# Autodesk Inventor assembly: Tower
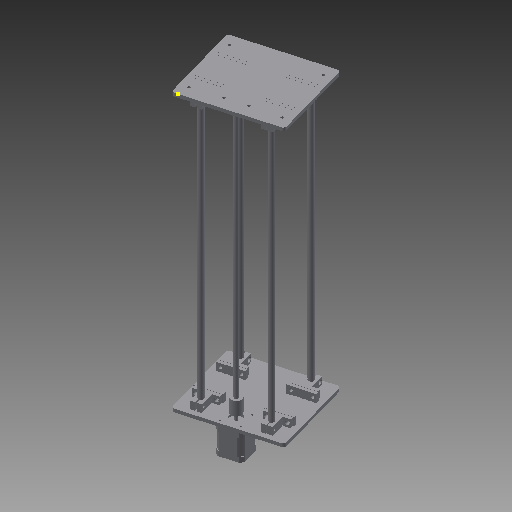
[picture p0: Inventor's stored thumbnail of the model, 512x512]
Saved by Autodesk Inventor 2019 (Build 230136000, 136)
## iProperties
Created: 2021-11-03
Part Number: Tower
Document SubType Name: Assembly
Designer: Mohamed
Author: Mohamed
## Documents named in this file (10)
- D:\mody\IndustrialLine\SortingAndStorage\Inventor\SSCARA Robot\Tower.iam
- D:\mody\IndustrialLine\SortingAndStorage\Inventor\SSCARA Robot\e_lead.ipt
- D:\mody\IndustrialLine\SortingAndStorage\Inventor\SSCARA Robot\e_coupler.ipt
- D:\mody\IndustrialLine\SortingAndStorage\Inventor\SSCARA Robot\e_circuler rod 400mm.ipt
- D:\mody\IndustrialLine\SortingAndStorage\Inventor\SSCARA Robot\e_top 1.ipt
- D:\mody\IndustrialLine\SortingAndStorage\Inventor\SSCARA Robot\e_linear rail support.ipt
- D:\mody\IndustrialLine\SortingAndStorage\Inventor\SSCARA Robot\nema 17 motor.ipt
- D:\mody\IndustrialLine\SortingAndStorage\Inventor\SSCARA Robot\e_rail support.ipt
- D:\mody\IndustrialLine\SortingAndStorage\Inventor\SSCARA Robot\e_k8_flanged bearing.iam
- D:\mody\IndustrialLine\SortingAndStorage\Inventor\SSCARA Robot\e_bot 1.ipt
## Components (26 placed, 9 different names)
1. e_top 1:1 — Mate:5, Mate:6, Mate:7, Mate:8, Mate:13, Flush:3, Flush:4, Flush:5, Flush:6, Mate:22, Mate:23, Mate:24, Mate:25, Mate:26, Mate:27, Mate:29, Mate:33, Mate:34, Mate:35, Mate:76, Mate:77
2. e_linear rail support:1 — Mate:5, Flush:1, Mate:14, Mate:19, Mate:30
3. e_linear rail support:2 — Mate:8, Flush:1, Mate:15, Mate:18, Mate:31
4. e_linear rail support:3 — Mate:7, Flush:2, Mate:17, Mate:21, Mate:32
5. e_linear rail support:4 — Mate:6, Flush:2, Mate:16, Mate:20, Mate:28
6. nema 17 motor:1 — Mate:13, Mate:38, Mate:39, Mate:76, Mate:77
7. e_rail support:1 — Flush:3, Mate:14, Mate:19, Mate:26, Mate:27
8. e_rail support:2 — Flush:4, Mate:15, Mate:18, Mate:25
9. e_rail support:3 — Flush:5, Mate:16, Mate:20, Mate:22, Mate:23
10. e_rail support:4 — Flush:6, Mate:17, Mate:21, Mate:24
11. e_circuler rod 400mm:1 — Mate:30, Mate:34, Mate:75
12. e_circuler rod 400mm:2 — Mate:31, Mate:33, Mate:79
13. e_circuler rod 400mm:3 — Mate:32, Mate:35, Mate:74
14. e_circuler rod 400mm:4 — Mate:28, Mate:29, Mate:73
15. e_coupler:1 — Mate:36, Mate:37, Mate:38
16. e_lead:1 — Mate:36, Mate:37, Mate:39, Mate:78
17. e_k8_flanged bearing:1 [sub-assembly] — Mate:68, Mate:69, Mate:70, Mate:78
18. e_bot 1:1 — Mate:40, Mate:41, Mate:42, Mate:43, Mate:44, Mate:45, Mate:46, Mate:47, Mate:48, Mate:49, Mate:50, Mate:51, Mate:68, Mate:69, Mate:70, Mate:79
19. e_rail support:5 — Mate:40, Mate:41, Mate:42, Mate:58, Mate:59, Mate:64
20. e_rail support:6 — Mate:49, Mate:50, Mate:51, Mate:60, Mate:61, Mate:67
21. e_rail support:7 — Mate:46, Mate:47, Mate:48, Mate:62, Mate:65, Mate:66
22. e_rail support:8 — Mate:43, Mate:44, Mate:45, Mate:52, Mate:53, Mate:63
23. e_linear rail support:5 — Mate:60, Mate:61, Mate:67, Mate:75
24. e_linear rail support:6 — Mate:58, Mate:59, Mate:64, Mate:73
25. e_linear rail support:7 — Mate:62, Mate:65, Mate:66
26. e_linear rail support:8 — Mate:52, Mate:53, Mate:63, Mate:74
## Relationships (71: Mate 65, Flush 6)
- Mate:5: e_top 1:1 ↔ e_linear rail support:1
- Mate:6: e_top 1:1 ↔ e_linear rail support:4
- Mate:7: e_top 1:1 ↔ e_linear rail support:3
- Mate:8: e_top 1:1 ↔ e_linear rail support:2
- Flush:1: e_linear rail support:1 ↔ e_linear rail support:2
- Flush:2: e_linear rail support:3 ↔ e_linear rail support:4
- Mate:13: e_top 1:1 ↔ nema 17 motor:1
- Flush:3: e_top 1:1 ↔ e_rail support:1
- Flush:4: e_top 1:1 ↔ e_rail support:2
- Flush:5: e_top 1:1 ↔ e_rail support:3
- Flush:6: e_top 1:1 ↔ e_rail support:4
- Mate:14: e_linear rail support:1 ↔ e_rail support:1
- Mate:15: e_linear rail support:2 ↔ e_rail support:2
- Mate:16: e_linear rail support:4 ↔ e_rail support:3
- Mate:17: e_linear rail support:3 ↔ e_rail support:4
- Mate:18: e_linear rail support:2 ↔ e_rail support:2
- Mate:19: e_linear rail support:1 ↔ e_rail support:1
- Mate:20: e_linear rail support:4 ↔ e_rail support:3
- Mate:21: e_linear rail support:3 ↔ e_rail support:4
- Mate:22: e_top 1:1 ↔ e_rail support:3
- Mate:23: e_top 1:1 ↔ e_rail support:3
- Mate:24: e_top 1:1 ↔ e_rail support:4
- Mate:25: e_top 1:1 ↔ e_rail support:2
- Mate:26: e_top 1:1 ↔ e_rail support:1
- Mate:27: e_top 1:1 ↔ e_rail support:1
- Mate:28: e_linear rail support:4 ↔ e_circuler rod 400mm:4
- Mate:29: e_top 1:1 ↔ e_circuler rod 400mm:4
- Mate:30: e_linear rail support:1 ↔ e_circuler rod 400mm:1
- Mate:31: e_linear rail support:2 ↔ e_circuler rod 400mm:2
- Mate:32: e_linear rail support:3 ↔ e_circuler rod 400mm:3
- Mate:33: e_top 1:1 ↔ e_circuler rod 400mm:2
- Mate:34: e_top 1:1 ↔ e_circuler rod 400mm:1
- Mate:35: e_top 1:1 ↔ e_circuler rod 400mm:3
- Mate:36: e_coupler:1 ↔ e_lead:1
- Mate:37: e_coupler:1 ↔ e_lead:1
- Mate:38: nema 17 motor:1 ↔ e_coupler:1
- Mate:39: nema 17 motor:1 ↔ e_lead:1
- Mate:40: e_bot 1:1 ↔ e_rail support:5
- Mate:41: e_bot 1:1 ↔ e_rail support:5
- Mate:42: e_bot 1:1 ↔ e_rail support:5
- Mate:43: e_bot 1:1 ↔ e_rail support:8
- Mate:44: e_bot 1:1 ↔ e_rail support:8
- Mate:45: e_bot 1:1 ↔ e_rail support:8
- Mate:46: e_bot 1:1 ↔ e_rail support:7
- Mate:47: e_bot 1:1 ↔ e_rail support:7
- Mate:48: e_bot 1:1 ↔ e_rail support:7
- Mate:49: e_bot 1:1 ↔ e_rail support:6
- Mate:50: e_bot 1:1 ↔ e_rail support:6
- Mate:51: e_bot 1:1 ↔ e_rail support:6
- Mate:52: e_rail support:8 ↔ e_linear rail support:8
- Mate:53: e_rail support:8 ↔ e_linear rail support:8
- Mate:58: e_rail support:5 ↔ e_linear rail support:6
- Mate:59: e_rail support:5 ↔ e_linear rail support:6
- Mate:60: e_rail support:6 ↔ e_linear rail support:5
- Mate:61: e_rail support:6 ↔ e_linear rail support:5
- Mate:62: e_rail support:7 ↔ e_linear rail support:7
- Mate:63: e_rail support:8 ↔ e_linear rail support:8
- Mate:64: e_rail support:5 ↔ e_linear rail support:6
- Mate:65: e_rail support:7 ↔ e_linear rail support:7
- Mate:66: e_rail support:7 ↔ e_linear rail support:7
- Mate:67: e_rail support:6 ↔ e_linear rail support:5
- Mate:68: e_k8_flanged bearing:1 ↔ e_bot 1:1
- Mate:69: e_k8_flanged bearing:1 ↔ e_bot 1:1
- Mate:70: e_k8_flanged bearing:1 ↔ e_bot 1:1
- Mate:73: e_circuler rod 400mm:4 ↔ e_linear rail support:6
- Mate:74: e_circuler rod 400mm:3 ↔ e_linear rail support:8
- Mate:75: e_circuler rod 400mm:1 ↔ e_linear rail support:5
- Mate:76: e_top 1:1 ↔ nema 17 motor:1
- Mate:77: e_top 1:1 ↔ nema 17 motor:1
- Mate:78: e_lead:1 ↔ e_k8_flanged bearing:1
- Mate:79: e_circuler rod 400mm:2 ↔ e_bot 1:1
